# Autodesk Inventor assembly: Przekładnia
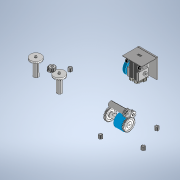
[picture p0: Inventor's stored thumbnail of the model, 180x180]
Saved by Autodesk Inventor 2022 (Build 260153000, 153)
## iProperties
Created: 2023-01-15
Part Number: Przekładnia
Document SubType Name: Assembly
Designer: komputer
Author: komputer
## Documents named in this file (22)
- D:\Inventor\NanoSumo\Przekładnia.iam
- D:\Inventor\NanoSumo\Moteur - Engrenage 4.ipt
- D:\Inventor\NanoSumo\Moteur - Engrenage 3.ipt
- D:\Inventor\NanoSumo\Moteur - Engrenage 2.ipt
- D:\Inventor\NanoSumo\Moteur - Engrenage 1.ipt
- D:\Inventor\NanoSumo\Moteur - Moteur.ipt
- D:\Inventor\NanoSumo\silnik_2.ipt
- C:\Users\komputer\Desktop\Moteur - Axe engrenage.ipt
- D:\Inventor\NanoSumo\kokool.ipt
- D:\Inventor\NanoSumo\lipol-40mAh.ipt
- D:\Inventor\NanoSumo\Przekładnia\Design Accelerator\Spur Gears2.iam
- D:\Inventor\NanoSumo\podłoga.ipt
- C:\Users\komputer\Desktop\Moteur - Engrenage 3_MIR1.ipt
- D:\Inventor\NanoSumo\ktir.ipt
- D:\Inventor\NanoSumo\ktir_MIR1.ipt
- D:\Inventor\NanoSumo\TOF_VL53L0X (1).ipt
- D:\Inventor\NanoSumo\Przekładnia\Design Accelerator\Spur Gears2_MIR1.iam
- D:\Inventor\NanoSumo\kokoko.ipt
- D:\Inventor\NanoSumo\elem.ipt
- D:\Inventor\NanoSumo\cos.ipt
- D:\Inventor\NanoSumo\pcb.ipt
- D:\Inventor\NanoSumo\przod.ipt
## Components (36 placed, 21 different names)
1. Moteur - Engrenage 2:1 — Mate:35, Mate:36
2. Moteur - Engrenage 1:1 — Mate:33, Mate:34, Flush:21, Flush:22
3. Moteur - Moteur:1
4. silnik_2:1 — Mate:21, Flush:6, Flush:7, Flush:17, Mate:30, Flush:25, Flush:28
5. silnik_2:2 — Mate:10, Mate:11
6. silnik_2:3 — Mate:20, Flush:4, Flush:5, Mate:21, Flush:6, Flush:7, Flush:24
7. Moteur - Engrenage 3:3 — Mate:10, Mate:11
8. silnik_2:4
9. Moteur - Engrenage 3:4
10. Moteur - Axe engrenage:2
11. Moteur - Axe engrenage:3
12. kokool:2 — Mate:26, Flush:11, Flush:18, Mate:42
13. lipol-40mAh:1 — Mate:40, Mate:41, Flush:26
14. Spur Gears:2 [sub-assembly] — Mate:30
15. Moteur - Engrenage 4:3
16. Moteur - Engrenage 4:4
17. Moteur - Moteur:2
18. podłoga:1 — Mate:20, Flush:4, Flush:5, Mate:24, Angle:1, Flush:11, Mate:28
19. Moteur - Engrenage 3:5 — Mate:42
20. Moteur - Engrenage 3_MIR1:1 — Mate:26
21. ktir:1 — Flush:17, Mate:28, Flush:18
22. ktir_MIR1:1
23. TOF_VL53L0X (1):1 — Flush:25, Mate:41
24. Spur Gears2_MIR1:1 [sub-assembly]
25. silnik_2:5 — Mate:35, Mate:36
26. Moteur - Moteur:3
27. Moteur - Engrenage 4:5
28. Moteur - Engrenage 1:2 — Mate:33, Mate:34, Flush:21
29. Moteur - Moteur:4
30. kokoko:1 — Flush:22
31. elem:1 — Flush:24, Mate:37, Mate:38, Mate:40
32. Moteur - Engrenage 3:6 — Mate:37, Mate:38, Mate:39
33. kokool:4 — Mate:39
34. cos:1 — Flush:26, Flush:27
35. pcb:1 — Flush:27
36. przod:1 — Flush:28
## Relationships (35: Mate 20, Flush 14, Angle 1)
- Mate:10: silnik_2:2 ↔ Moteur - Engrenage 3:3
- Mate:11: silnik_2:2 ↔ Moteur - Engrenage 3:3
- [Mate]: silnik_2:4 ↔ Moteur - Engrenage 3:4
- [Mate]: silnik_2:4 ↔ Moteur - Engrenage 3:4
- Mate:20: silnik_2:3 ↔ podłoga:1
- Flush:4: silnik_2:3 ↔ podłoga:1
- Flush:5: silnik_2:3 ↔ podłoga:1
- Mate:21: silnik_2:1 ↔ silnik_2:3
- Flush:6: silnik_2:1 ↔ silnik_2:3
- Flush:7: silnik_2:1 ↔ silnik_2:3
- Mate:24: podłoga:1
- Angle:1 (0 deg): podłoga:1
- Mate:26: kokool:2 ↔ Moteur - Engrenage 3_MIR1:1
- Flush:11: kokool:2 ↔ podłoga:1
- Flush:17 (2 mm): silnik_2:1 ↔ ktir:1
- Mate:28 (5 mm): podłoga:1 ↔ ktir:1
- Flush:18 (-3 mm): kokool:2 ↔ ktir:1
- Mate:30 (0.1 mm): silnik_2:1 ↔ Spur Gears:2
- Mate:33: Moteur - Engrenage 1:1 ↔ Moteur - Engrenage 1:2
- Mate:34: Moteur - Engrenage 1:1 ↔ Moteur - Engrenage 1:2
- Flush:21: Moteur - Engrenage 1:1 ↔ Moteur - Engrenage 1:2
- Mate:35: Moteur - Engrenage 2:1 ↔ silnik_2:5
- Mate:36: Moteur - Engrenage 2:1 ↔ silnik_2:5
- Flush:22: Moteur - Engrenage 1:1 ↔ kokoko:1
- Flush:24: silnik_2:3 ↔ elem:1
- Mate:37: elem:1 ↔ Moteur - Engrenage 3:6
- Mate:38 (0.3 mm): elem:1 ↔ Moteur - Engrenage 3:6
- Mate:39: Moteur - Engrenage 3:6 ↔ kokool:4
- Flush:25: silnik_2:1 ↔ TOF_VL53L0X (1):1
- Mate:40 (1.5 mm): lipol-40mAh:1 ↔ elem:1
- Mate:41: lipol-40mAh:1 ↔ TOF_VL53L0X (1):1
- Flush:26: lipol-40mAh:1 ↔ cos:1
- Flush:27: cos:1 ↔ pcb:1
- Flush:28: silnik_2:1 ↔ przod:1
- Mate:42: kokool:2 ↔ Moteur - Engrenage 3:5
## Named parameters: d12_d10 = 0 mm, d13_d11 = 0 mm
